# Autodesk Inventor assembly: exhaustFilterHousing
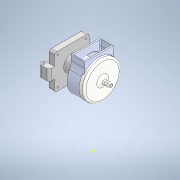
[picture p0: Inventor's stored thumbnail of the model, 180x180]
Saved by Autodesk Inventor 2020 (Build 240168000, 168)
## iProperties
Created: 2020-04-09
Part Number: exhaustFilterHousing
Document SubType Name: Assembly
Designer: Simon
Author: Simon
## Documents named in this file (4)
- \\Mac\Home\Desktop\3D\Breeze thing\Filter housing with o ring\exhaustFilterHousing.iam
- \\Mac\Home\Desktop\3D\Breeze thing\Filter housing with o ring\exhaustboy.ipt
- \\Mac\Home\Desktop\3D\Breeze thing\Filter housing with o ring\check valve v2 v1.ipt
- \\Mac\Home\Desktop\3D\Breeze thing\Filter housing with o ring\exhaustCap.ipt
## Components (3 placed, 3 different names)
1. exhaustboy:1 — Mate:1, Mate:2, Angle:1, Mate:3, Mate:4
2. check valve v2 v1:1 — Mate:1, Mate:2, Angle:1
3. exhaustCap:1 — Mate:3, Mate:4
## Relationships (5: Mate 4, Angle 1)
- Mate:1: exhaustboy:1 ↔ check valve v2 v1:1
- Mate:2: exhaustboy:1 ↔ check valve v2 v1:1
- Angle:1 (180 deg): exhaustboy:1 ↔ check valve v2 v1:1
- Mate:3: exhaustboy:1 ↔ exhaustCap:1
- Mate:4: exhaustboy:1 ↔ exhaustCap:1
